# Autodesk Inventor assembly: FullAssembly
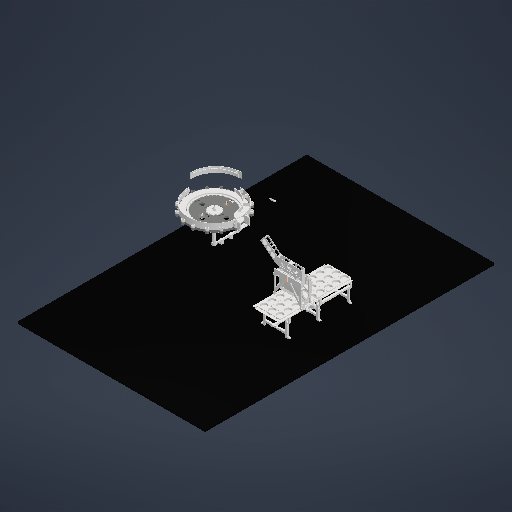
[picture p0: Inventor's stored thumbnail of the model, 512x512]
Saved by Autodesk Inventor 2026 (Build 300175050, 175E)
## iProperties
Created: 2026-05-08
Part Number: FullAssembly
Document SubType Name: Assembly
Designer: sniel
Author: sniel
## Documents named in this file (4)
- C:\Users\sniel\OneDrive\SDU\4_Semester\Applied automation\AppliedAutomationProject\feeder\FullAssembly.iam
- C:\Users\sniel\OneDrive\SDU\4_Semester\Applied automation\AppliedAutomationProject\feeder\FeederV3.iam
- C:\Users\sniel\OneDrive\SDU\4_Semester\Applied automation\AppliedAutomationProject\feeder\trayFeeder\TrayFeeder.iam
- C:\Users\sniel\OneDrive\SDU\4_Semester\Applied automation\AppliedAutomationProject\feeder\table.ipt
## Components (3 placed, 3 different names)
1. FeederV3:1 [sub-assembly]
2. TrayFeeder:1 [sub-assembly] — Mate:1
3. table:1 — Mate:1
## Relationships (1: Mate 1)
- Mate:1: TrayFeeder:1 ↔ table:1
